# Autodesk Inventor assembly: LF
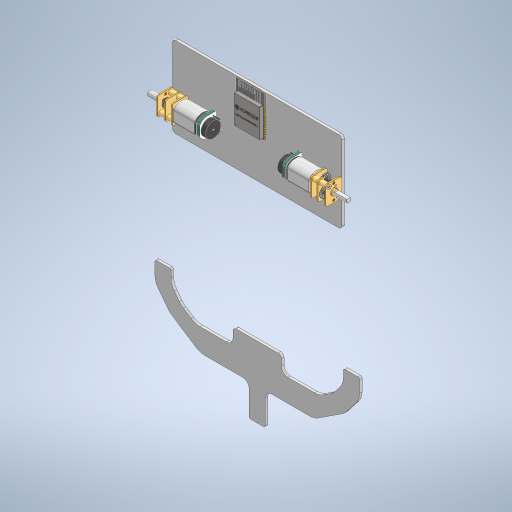
[picture p0: Inventor's stored thumbnail of the model, 512x512]
Saved by Autodesk Inventor 2023 (Build 270158000, 158)
## iProperties
Created: 2024-03-30
Part Number: LF
Document SubType Name: Assembly
Designer: Kamil
Author: Kamil
## Documents named in this file (6)
- C:\Users\Kamil\Documents\Inventor\LF_1\LF.iam
- C:\Users\Kamil\Documents\Inventor\LF_1\przód.ipt
- C:\Users\Kamil\Documents\Inventor\LF_1\QRE1113GR.ipt
- C:\Users\Kamil\Documents\Inventor\LF_1\ty.ipt
- C:\Users\Kamil\Documents\Inventor\LF_1\N20 Mini Micro Metall Gear Motor DC 3-6-12V v1.ipt
- C:\Users\Kamil\Documents\Inventor\LF_1\ESP32-S3-WROOM-1.ipt
## Components (11 placed, 5 different names)
1. przód:1 — Równoległe:8, Równoległe:9, Zestawiające:9, Równoległe:10, Zestawiające:10, Równoległe:11, Zestawiające:11, Równoległe:12
2. QRE1113GR:1 — Równoległe:3, Równoległe:5, Zestawiające:6, Równoległe:8, Równoległe:9
3. QRE1113GR:10 — Zestawiające:5, Równoległe:2
4. QRE1113GR:11 — Zestawiające:5, Równoległe:2
5. QRE1113GR:12 — Równoległe:3, Równoległe:4, Równoległe:5, Równoległe:6, Zestawiające:6, Zestawiające:7
6. QRE1113GR:13 — Równoległe:4, Równoległe:6, Zestawiające:7
7. QRE1113GR:14 — Zestawiające:9, Równoległe:10, Zestawiające:10
8. ty:1 — Równoległe:11, Zestawiające:11, Równoległe:12, Zestawiające:12, Zestawiające:13, Równoległe:13, Równoległe:14, Zestawiające:14, Równoległe:15
9. N20 Mini Micro Metall Gear Motor DC 3-6-12V v1:1 — Zestawiające:13, Równoległe:13
10. N20 Mini Micro Metall Gear Motor DC 3-6-12V v1:2 — Zestawiające:12, Równoległe:14
11. ESP32-S3-WROOM-1:1 — Zestawiające:14, Równoległe:15
## Relationships (22: Flush 13, Mate 9)
- Zestawiające:5 [Mate] (5 mm): QRE1113GR:10 ↔ QRE1113GR:11
- Równoległe:2 [Flush] (10 mm): QRE1113GR:10 ↔ QRE1113GR:11
- Równoległe:3 [Flush]: QRE1113GR:1 ↔ QRE1113GR:12
- Równoległe:4 [Flush]: QRE1113GR:12 ↔ QRE1113GR:13
- Równoległe:5 [Flush] (-7 mm): QRE1113GR:1 ↔ QRE1113GR:12
- Równoległe:6 [Flush] (-10 mm): QRE1113GR:12 ↔ QRE1113GR:13
- Zestawiające:6 [Mate] (8 mm): QRE1113GR:1 ↔ QRE1113GR:12
- Zestawiające:7 [Mate] (5 mm): QRE1113GR:12 ↔ QRE1113GR:13
- Równoległe:8 [Flush] (3.3 mm): przód:1 ↔ QRE1113GR:1
- Równoległe:9 [Flush] (-5.15 mm): przód:1 ↔ QRE1113GR:1
- Zestawiające:9 [Mate]: przód:1 ↔ QRE1113GR:14
- Równoległe:10 [Flush] (2 mm): przód:1 ↔ QRE1113GR:14
- Zestawiające:10 [Mate] (-3.65 mm): przód:1 ↔ QRE1113GR:14
- Równoległe:11 [Flush]: przód:1 ↔ ty:1
- Zestawiające:11 [Mate] (-180 mm): przód:1 ↔ ty:1
- Równoległe:12 [Flush] (-10.925 mm): przód:1 ↔ ty:1
- Zestawiające:12 [Mate]: ty:1 ↔ N20 Mini Micro Metall Gear Motor DC 3-6-12V v1:2
- Zestawiające:13 [Mate]: ty:1 ↔ N20 Mini Micro Metall Gear Motor DC 3-6-12V v1:1
- Równoległe:13 [Flush]: ty:1 ↔ N20 Mini Micro Metall Gear Motor DC 3-6-12V v1:1
- Równoległe:14 [Flush]: ty:1 ↔ N20 Mini Micro Metall Gear Motor DC 3-6-12V v1:2
- Zestawiające:14 [Mate]: ty:1 ↔ ESP32-S3-WROOM-1:1
- Równoległe:15 [Flush]: ty:1 ↔ ESP32-S3-WROOM-1:1
